# Autodesk Inventor assembly: Shooting Mechanism Assembly FINAL 2
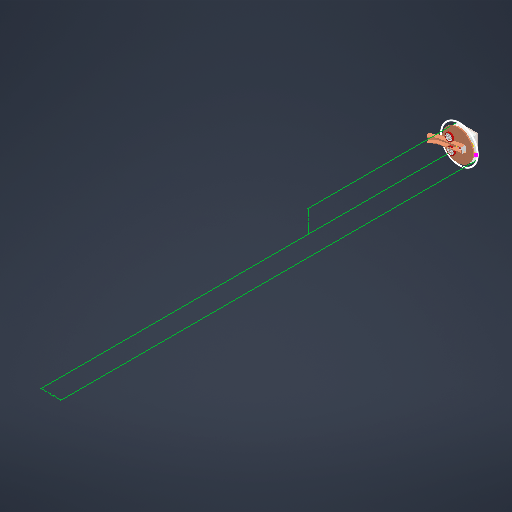
[picture p0: Inventor's stored thumbnail of the model, 512x512]
Saved by Autodesk Inventor 2026.2 (Build 302298000, 298)
## iProperties
Created: 2026-04-15
Part Number: Shooting Mechanism Assembly FINAL 2
Document SubType Name: Assembly
Designer: yassi
Author: yassi
## Documents named in this file (13)
- C:\Users\danda\BOM-project\Project\CAD\Shooting\Shooting Mechanism Assembly FINAL 2.iam
- C:\Users\danda\BOM-project\Project\CAD\Shooting\arduinouno.ipt
- C:\Users\danda\BOM-project\Project\CAD\Shooting\Assembly1.iam
- C:\Users\danda\BOM-project\Project\CAD\Shooting\flywheel.ipt
- C:\Users\danda\BOM-project\Project\CAD\Shooting\H-brug.ipt
- C:\Users\danda\BOM-project\Project\CAD\Shooting\MG_996R.iam
- C:\Users\danda\BOM-project\Project\CAD\Shooting\Mini Push Pull Solenoid 4mm.ipt
- C:\Users\danda\BOM-project\Project\CAD\Shooting\Rotating Base.ipt
- C:\Users\danda\BOM-project\Project\CAD\Shooting\Servo Mount.ipt
- C:\Users\danda\BOM-project\Project\CAD\Shooting\Servo Stand.ipt
- C:\Users\danda\BOM-project\Project\CAD\Shooting\Shooting Mechanism Box.ipt
- C:\Users\danda\BOM-project\Project\CAD\Shooting\Shooting Ramp.ipt
- C:\Users\danda\BOM-project\Project\CAD\Shooting\Part7.ipt
## Components (14 placed, 12 different names)
1. Assembly1:1 [sub-assembly] — Mate:16, Mate:18, Mate:19, Mate:20, Mate:21, Mate:33, Insert:2, Mate:38
2. flywheel:1 — Mate:33, Insert:2
3. H-brug:1 — Mate:43, Mate:44, Mate:45
4. MG_996R:1 [sub-assembly] — Mate:13, Mate:14, Mate:15, Insert:4
5. Mini Push Pull Solenoid 4mm:1 — Mate:30, Mate:31, Mate:34
6. Rotating Base:1 — Mate:16, Mate:17, Mate:18, Mate:19, Mate:20, Mate:21, Mate:23, Mate:24, Mate:25, Mate:26, Mate:27, Mate:28, Mate:29, Mate:35, Mate:38, Mate:49, Insert:3
7. Servo Mount:1 — Mate:10, Mate:11, Mate:12, Mate:13, Mate:14, Mate:15
8. Servo Stand:1 — Mate:10, Mate:11, Mate:12, Mate:46, Mate:47, Mate:48
9. Shooting Mechanism Box:1 — Mate:41, Mate:42, Mate:43, Mate:44, Mate:45, Mate:46, Mate:47, Mate:48, Mate:51, Mate:52, Mate:53
10. Shooting Ramp:1 — Mate:28, Mate:29, Mate:30, Mate:31, Mate:34, Mate:35
11. arduinouno:1 — Mate:41, Mate:42
12. Assembly1:2 [sub-assembly] — Mate:17, Mate:23, Mate:24, Mate:25, Mate:26, Mate:27, Mate:32, Mate:36, Mate:37
13. flywheel:2 — Mate:32, Mate:36, Mate:37
14. Part7:1 — Mate:49, Insert:3, Insert:4
## Relationships (43: Mate 40, Insert 3)
- Mate:10: Servo Mount:1 ↔ Servo Stand:1
- Mate:11: Servo Mount:1 ↔ Servo Stand:1
- Mate:12: Servo Mount:1 ↔ Servo Stand:1
- Mate:13: MG_996R:1 ↔ Servo Mount:1
- Mate:14: MG_996R:1 ↔ Servo Mount:1
- Mate:15: MG_996R:1 ↔ Servo Mount:1
- Mate:16: Assembly1:1 ↔ Rotating Base:1
- Mate:17: Rotating Base:1 ↔ Assembly1:2
- Mate:18: Assembly1:1 ↔ Rotating Base:1
- Mate:19: Assembly1:1 ↔ Rotating Base:1
- Mate:20: Assembly1:1 ↔ Rotating Base:1
- Mate:21: Assembly1:1 ↔ Rotating Base:1
- Mate:23: Rotating Base:1 ↔ Assembly1:2
- Mate:24: Rotating Base:1 ↔ Assembly1:2
- Mate:25: Rotating Base:1 ↔ Assembly1:2
- Mate:26: Rotating Base:1 ↔ Assembly1:2
- Mate:27: Rotating Base:1 ↔ Assembly1:2
- Mate:28: Rotating Base:1 ↔ Shooting Ramp:1
- Mate:29: Rotating Base:1 ↔ Shooting Ramp:1
- Mate:30: Mini Push Pull Solenoid 4mm:1 ↔ Shooting Ramp:1
- Mate:31 (5 mm): Mini Push Pull Solenoid 4mm:1 ↔ Shooting Ramp:1
- Mate:32: Assembly1:2 ↔ flywheel:2
- Mate:33: Assembly1:1 ↔ flywheel:1
- Mate:34: Mini Push Pull Solenoid 4mm:1 ↔ Shooting Ramp:1
- Insert:2: Assembly1:1 ↔ flywheel:1
- Mate:35: Rotating Base:1 ↔ Shooting Ramp:1
- Mate:36: Assembly1:2 ↔ flywheel:2
- Mate:37: Assembly1:2 ↔ flywheel:2
- Mate:38: Assembly1:1 ↔ Rotating Base:1
- Mate:41: Shooting Mechanism Box:1 ↔ arduinouno:1
- Mate:42: Shooting Mechanism Box:1 ↔ arduinouno:1
- Mate:43: H-brug:1 ↔ Shooting Mechanism Box:1
- Mate:44: H-brug:1 ↔ Shooting Mechanism Box:1
- Mate:45: H-brug:1 ↔ Shooting Mechanism Box:1
- Mate:46: Servo Stand:1 ↔ Shooting Mechanism Box:1
- Mate:47: Servo Stand:1 ↔ Shooting Mechanism Box:1
- Mate:48: Servo Stand:1 ↔ Shooting Mechanism Box:1
- Mate:49: Rotating Base:1 ↔ Part7:1
- Insert:3: Rotating Base:1 ↔ Part7:1
- Insert:4: MG_996R:1 ↔ Part7:1
- Mate:51: Shooting Mechanism Box:1
- Mate:52: Shooting Mechanism Box:1
- Mate:53: Shooting Mechanism Box:1
## Named parameters: Finish1_Area = 70.7173
note: some values were not read from the file. Shown as the stored number, unit unknown: "Finish1_Area".
